# Autodesk Inventor assembly: RAI_Assembly
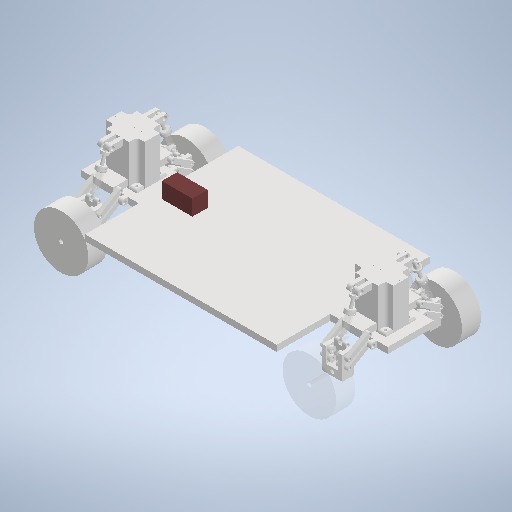
[picture p0: Inventor's stored thumbnail of the model, 512x512]
Saved by Autodesk Inventor 2025.2 (Build 292293000, 293)
## iProperties
Created: 2025-01-03
Part Number: RAI_Assembly
Document SubType Name: Assembly
Designer: SEON
Author: SEON
## Documents named in this file (15)
- C:\Users\SEON\Documents\Inventor\ProjectRAI\RAI_Assembly.iam
- C:\Users\SEON\Documents\Inventor\ProjectRAI\BottomFrame.ipt
- C:\Users\SEON\Documents\Inventor\ProjectRAI\SuspensionSupporter.ipt
- C:\Users\SEON\Documents\Inventor\ProjectRAI\TireDummy.ipt
- C:\Users\SEON\Documents\Inventor\ProjectRAI\SteeringFrame.ipt
- C:\Users\SEON\Documents\Inventor\ProjectRAI\SteeringConnector.ipt
- C:\Users\SEON\Documents\Inventor\ProjectRAI\SuspensionFrame.ipt
- C:\Users\SEON\Documents\Inventor\ProjectRAI\SuspensionAssembly.iam
- C:\Users\SEON\Documents\Inventor\ProjectRAI\SteeringFrameFront.ipt
- C:\Users\SEON\Documents\Inventor\ProjectRAI\Steering.ipt
- C:\Users\SEON\Documents\Inventor\ProjectRAI\996R_Servo.ipt
- C:\Users\SEON\Documents\Inventor\ProjectRAI\SteeringBase.ipt
- C:\Users\SEON\Documents\Inventor\ProjectRAI\SteeringAxis.ipt
- C:\Users\SEON\Documents\Inventor\ProjectRAI\DummyBallJoint.ipt
- C:\Users\SEON\Documents\Inventor\ProjectRAI\DummyBallJointF.ipt
## Components (64 placed, 14 different names)
1. BottomFrame:1 — 메이트:1, 메이트:2, 메이트:3, 메이트:5, 메이트:6, 메이트:17, 메이트:18, 메이트:21, 메이트:37, 메이트:43, 메이트:55, 메이트:62, 메이트:63, 메이트:64, 메이트:65, 메이트:67, 메이트:89, 메이트:91, 메이트:93, 메이트:111, 메이트:113, 메이트:115, 메이트:130, 메이트:152, 메이트:153, 메이트:154
2. SuspensionSupporter:1 — 메이트:1, 메이트:2, 메이트:3, 메이트:4, 메이트:46, 메이트:56, 메이트:146, 메이트:147, 메이트:149, 메이트:151
3. SuspensionSupporter:2 — 메이트:4, 메이트:5, 메이트:6, 메이트:23, 메이트:26, 메이트:35
4. TireDummy:1 — 메이트:7, 메이트:8
5. SteeringFrame:1 — 메이트:7, 메이트:8, 메이트:9, 메이트:10, 메이트:11, 메이트:12, 메이트:19, 메이트:24, 메이트:27, 메이트:28, 메이트:29, 메이트:30, 메이트:33, 메이트:34
6. SuspensionFrame:2 — 메이트:13, 메이트:14, 메이트:18, 메이트:21
7. SteeringConnector:3 — 메이트:9, 메이트:10, 메이트:13, 메이트:14
8. SteeringConnector:4 — 메이트:11, 메이트:12, 메이트:15, 메이트:16
9. SuspensionFrame:3 — 메이트:15, 메이트:16, 메이트:17
10. SuspensionFrame:4 — 메이트:19, 메이트:23, 메이트:31
11. SuspensionFrame:5 — 메이트:24, 메이트:26, 메이트:32
12. SteeringConnector:5 — 메이트:27, 메이트:28, 메이트:32
13. SteeringConnector:6 — 메이트:29, 메이트:30, 메이트:31
14. SuspensionAssembly:1 [sub-assembly] — 메이트:33, 메이트:34, 메이트:35
15. SuspensionFrame:6 — 메이트:44, 메이트:45, 메이트:46
16. SuspensionFrame:7 — 메이트:53, 메이트:54, 메이트:55
17. SuspensionFrame:8 — 메이트:36, 메이트:37, 메이트:42, 메이트:43
18. SuspensionFrame:9 — 메이트:51, 메이트:52, 메이트:56
19. SteeringFrame:2 — 메이트:36, 메이트:38, 메이트:39, 메이트:40, 메이트:41, 메이트:45, 메이트:47, 메이트:48, 메이트:49, 메이트:50, 메이트:60, 메이트:61, 메이트:148, 메이트:150
20. SteeringConnector:7 — 메이트:48, 메이트:49, 메이트:51, 메이트:52
21. SteeringConnector:8 — 메이트:38, 메이트:39, 메이트:44
22. SteeringConnector:9 — 메이트:47, 메이트:50, 메이트:53, 메이트:54
23. SteeringConnector:10 — 메이트:40, 메이트:41, 메이트:42
24. TireDummy:2 — 메이트:60, 메이트:61
25. SuspensionSupporter:3 — 메이트:62, 메이트:66, 메이트:67, 메이트:68, 메이트:69, 메이트:90, 메이트:92, 메이트:131
26. SuspensionSupporter:4 — 메이트:63, 메이트:64, 메이트:65, 메이트:66, 메이트:70, 메이트:71, 메이트:112, 메이트:114, 메이트:135, 메이트:136
27. SuspensionAssembly:3 [sub-assembly] — 메이트:68, 메이트:69, 메이트:129
28. SuspensionAssembly:4 [sub-assembly] — 메이트:70, 메이트:71, 메이트:125
29. SuspensionFrame:10 — 메이트:84, 메이트:85, 메이트:93, 메이트:127, 메이트:130
30. SuspensionFrame:11 — 메이트:82, 메이트:83, 메이트:90, 메이트:133
31. SuspensionFrame:12 — 메이트:86, 메이트:87, 메이트:92, 메이트:128, 메이트:131
32. SuspensionFrame:13 — 메이트:80, 메이트:81, 메이트:89, 메이트:91
33. SteeringConnector:11 — 메이트:86, 메이트:87
34. SteeringConnector:12 — 메이트:84, 메이트:85, 메이트:126
35. SteeringConnector:13 — 메이트:82, 메이트:83, 메이트:132
36. SteeringConnector:14 — 메이트:80, 메이트:81, 메이트:134
37. SuspensionFrame:14 — 메이트:113, 메이트:137
38. SuspensionFrame:15 — 메이트:112, 메이트:121, 메이트:135
39. SuspensionFrame:16 — 메이트:114, 메이트:136
40. SuspensionFrame:17 — 메이트:111, 메이트:115, 메이트:122
41. SteeringConnector:15 — 메이트:124
42. SteeringConnector:16 — 메이트:123
43. SteeringConnector:17 — 메이트:120
44. SteeringConnector:18
45. TireDummy:3 — 메이트:143, 메이트:144
46. TireDummy:4 — 메이트:140, 메이트:141
47. SteeringFrameFront:1 — 메이트:120, 메이트:121, 메이트:122, 메이트:123, 메이트:124, 메이트:125, 메이트:137, 메이트:142, 메이트:145
48. SteeringFrameFront:2 — 메이트:126, 메이트:127, 메이트:128, 메이트:129, 메이트:132, 메이트:133, 메이트:134, 메이트:138, 메이트:139
49. Steering:1 — 메이트:138, 메이트:139, 메이트:140, 메이트:141, 메이트:167, 메이트:168
50. Steering:2 — 메이트:142, 메이트:143, 메이트:144, 메이트:145, 메이트:165, 메이트:166
51. SuspensionAssembly:5 [sub-assembly] — 메이트:146, 메이트:147, 메이트:148
52. SuspensionAssembly:6 [sub-assembly] — 메이트:149, 메이트:150, 메이트:151
53. 996R_Servo:1 — 메이트:152, 메이트:153, 메이트:154, 메이트:155, 메이트:156
54. SteeringBase:1 — 메이트:155, 메이트:156, 메이트:161, 메이트:162, 메이트:163, 메이트:164
55. DummyBallJoint:1 — 메이트:161, 메이트:162, 접선:2
56. DummyBallJoint:2 — 메이트:163, 메이트:164, 접선:3
57. DummyBallJointF:1 — 메이트:169, 메이트:172, 접선:2
58. DummyBallJointF:2 — 메이트:170, 메이트:171, 접선:1
59. DummyBallJoint:3 — 메이트:165, 메이트:166, 접선:1
60. DummyBallJoint:4 — 메이트:167, 메이트:168, 접선:4
61. SteeringAxis:4 — 메이트:169, 메이트:170, 메이트:171, 메이트:172
62. DummyBallJointF:3 — 접선:4
63. DummyBallJointF:4 — 접선:3
64. SteeringAxis:5
## Relationships (148: Mate 144, Tangent 4)
- 메이트:1 [Mate]: BottomFrame:1 ↔ SuspensionSupporter:1
- 메이트:2 [Mate]: BottomFrame:1 ↔ SuspensionSupporter:1
- 메이트:3 [Mate]: BottomFrame:1 ↔ SuspensionSupporter:1
- 메이트:4 [Mate]: SuspensionSupporter:1 ↔ SuspensionSupporter:2
- 메이트:5 [Mate]: BottomFrame:1 ↔ SuspensionSupporter:2
- 메이트:6 [Mate]: BottomFrame:1 ↔ SuspensionSupporter:2
- 메이트:7 [Mate]: TireDummy:1 ↔ SteeringFrame:1
- 메이트:8 [Mate] (5 mm): TireDummy:1 ↔ SteeringFrame:1
- 메이트:9 [Mate]: SteeringFrame:1 ↔ SteeringConnector:3
- 메이트:10 [Mate]: SteeringFrame:1 ↔ SteeringConnector:3
- 메이트:11 [Mate]: SteeringFrame:1 ↔ SteeringConnector:4
- 메이트:12 [Mate]: SteeringFrame:1 ↔ SteeringConnector:4
- 메이트:13 [Mate]: SuspensionFrame:2 ↔ SteeringConnector:3
- 메이트:14 [Mate]: SuspensionFrame:2 ↔ SteeringConnector:3
- 메이트:15 [Mate]: SteeringConnector:4 ↔ SuspensionFrame:3
- 메이트:16 [Mate]: SteeringConnector:4 ↔ SuspensionFrame:3
- 메이트:17 [Mate]: BottomFrame:1 ↔ SuspensionFrame:3
- 메이트:18 [Mate]: BottomFrame:1 ↔ SuspensionFrame:2
- 메이트:19 [Mate]: SteeringFrame:1 ↔ SuspensionFrame:4
- 메이트:21 [Mate]: BottomFrame:1 ↔ SuspensionFrame:2
- 메이트:23 [Mate]: SuspensionSupporter:2 ↔ SuspensionFrame:4
- 메이트:24 [Mate]: SteeringFrame:1 ↔ SuspensionFrame:5
- 메이트:26 [Mate]: SuspensionSupporter:2 ↔ SuspensionFrame:5
- 메이트:27 [Mate]: SteeringFrame:1 ↔ SteeringConnector:5
- 메이트:28 [Mate]: SteeringFrame:1 ↔ SteeringConnector:5
- 메이트:29 [Mate]: SteeringFrame:1 ↔ SteeringConnector:6
- 메이트:30 [Mate]: SteeringFrame:1 ↔ SteeringConnector:6
- 메이트:31 [Mate]: SuspensionFrame:4 ↔ SteeringConnector:6
- 메이트:32 [Mate]: SuspensionFrame:5 ↔ SteeringConnector:5
- 메이트:33 [Mate]: SteeringFrame:1 ↔ SuspensionAssembly:1
- 메이트:34 [Mate]: SteeringFrame:1 ↔ SuspensionAssembly:1
- 메이트:35 [Mate]: SuspensionSupporter:2 ↔ SuspensionAssembly:1
- 메이트:36 [Mate]: SuspensionFrame:8 ↔ SteeringFrame:2
- 메이트:37 [Mate]: BottomFrame:1 ↔ SuspensionFrame:8
- 메이트:38 [Mate]: SteeringFrame:2 ↔ SteeringConnector:8
- 메이트:39 [Mate]: SteeringFrame:2 ↔ SteeringConnector:8
- 메이트:40 [Mate]: SteeringFrame:2 ↔ SteeringConnector:10
- 메이트:41 [Mate]: SteeringFrame:2 ↔ SteeringConnector:10
- 메이트:42 [Mate]: SuspensionFrame:8 ↔ SteeringConnector:10
- 메이트:43 [Mate]: BottomFrame:1 ↔ SuspensionFrame:8
- 메이트:44 [Mate]: SuspensionFrame:6 ↔ SteeringConnector:8
- 메이트:45 [Mate]: SuspensionFrame:6 ↔ SteeringFrame:2
- 메이트:46 [Mate]: SuspensionSupporter:1 ↔ SuspensionFrame:6
- 메이트:47 [Mate]: SteeringFrame:2 ↔ SteeringConnector:9
- 메이트:48 [Mate]: SteeringFrame:2 ↔ SteeringConnector:7
- 메이트:49 [Mate]: SteeringFrame:2 ↔ SteeringConnector:7
- 메이트:50 [Mate]: SteeringFrame:2 ↔ SteeringConnector:9
- 메이트:51 [Mate]: SuspensionFrame:9 ↔ SteeringConnector:7
- 메이트:52 [Mate]: SuspensionFrame:9 ↔ SteeringConnector:7
- 메이트:53 [Mate]: SuspensionFrame:7 ↔ SteeringConnector:9
- 메이트:54 [Mate]: SuspensionFrame:7 ↔ SteeringConnector:9
- 메이트:55 [Mate]: BottomFrame:1 ↔ SuspensionFrame:7
- 메이트:56 [Mate]: SuspensionSupporter:1 ↔ SuspensionFrame:9
- 메이트:60 [Mate]: SteeringFrame:2 ↔ TireDummy:2
- 메이트:61 [Mate] (5 mm): SteeringFrame:2 ↔ TireDummy:2
- 메이트:62 [Mate]: BottomFrame:1 ↔ SuspensionSupporter:3
- 메이트:63 [Mate]: BottomFrame:1 ↔ SuspensionSupporter:4
- 메이트:64 [Mate]: BottomFrame:1 ↔ SuspensionSupporter:4
- 메이트:65 [Mate]: BottomFrame:1 ↔ SuspensionSupporter:4
- 메이트:66 [Mate]: SuspensionSupporter:3 ↔ SuspensionSupporter:4
- 메이트:67 [Mate]: BottomFrame:1 ↔ SuspensionSupporter:3
- 메이트:68 [Mate]: SuspensionSupporter:3 ↔ SuspensionAssembly:3
- 메이트:69 [Mate]: SuspensionSupporter:3 ↔ SuspensionAssembly:3
- 메이트:70 [Mate]: SuspensionSupporter:4 ↔ SuspensionAssembly:4
- 메이트:71 [Mate]: SuspensionSupporter:4 ↔ SuspensionAssembly:4
- 메이트:80 [Mate]: SuspensionFrame:13 ↔ SteeringConnector:14
- 메이트:81 [Mate]: SuspensionFrame:13 ↔ SteeringConnector:14
- 메이트:82 [Mate]: SuspensionFrame:11 ↔ SteeringConnector:13
- 메이트:83 [Mate]: SuspensionFrame:11 ↔ SteeringConnector:13
- 메이트:84 [Mate]: SuspensionFrame:10 ↔ SteeringConnector:12
- 메이트:85 [Mate]: SuspensionFrame:10 ↔ SteeringConnector:12
- 메이트:86 [Mate]: SuspensionFrame:12 ↔ SteeringConnector:11
- 메이트:87 [Mate]: SuspensionFrame:12 ↔ SteeringConnector:11
- 메이트:89 [Mate]: BottomFrame:1 ↔ SuspensionFrame:13
- 메이트:90 [Mate]: SuspensionSupporter:3 ↔ SuspensionFrame:11
- 메이트:91 [Mate]: BottomFrame:1 ↔ SuspensionFrame:13
- 메이트:92 [Mate]: SuspensionSupporter:3 ↔ SuspensionFrame:12
- 메이트:93 [Mate]: BottomFrame:1 ↔ SuspensionFrame:10
- [Mate]: SuspensionFrame:17 ↔ SteeringConnector:18
- [Mate]: SuspensionFrame:17 ↔ SteeringConnector:18
- [Mate]: SuspensionFrame:15 ↔ SteeringConnector:17
- [Mate]: SuspensionFrame:15 ↔ SteeringConnector:17
- [Mate]: SuspensionFrame:14 ↔ SteeringConnector:16
- [Mate]: SuspensionFrame:14 ↔ SteeringConnector:16
- [Mate]: SuspensionFrame:16 ↔ SteeringConnector:15
- [Mate]: SuspensionFrame:16 ↔ SteeringConnector:15
- 메이트:111 [Mate]: BottomFrame:1 ↔ SuspensionFrame:17
- 메이트:112 [Mate]: SuspensionSupporter:4 ↔ SuspensionFrame:15
- 메이트:113 [Mate]: BottomFrame:1 ↔ SuspensionFrame:14
- 메이트:114 [Mate]: SuspensionSupporter:4 ↔ SuspensionFrame:16
- 메이트:115 [Mate]: BottomFrame:1 ↔ SuspensionFrame:17
- 메이트:120 [Mate]: SteeringConnector:17 ↔ SteeringFrameFront:1
- 메이트:121 [Mate]: SuspensionFrame:15 ↔ SteeringFrameFront:1
- 메이트:122 [Mate]: SuspensionFrame:17 ↔ SteeringFrameFront:1
- 메이트:123 [Mate]: SteeringConnector:16 ↔ SteeringFrameFront:1
- 메이트:124 [Mate]: SteeringConnector:15 ↔ SteeringFrameFront:1
- 메이트:125 [Mate]: SuspensionAssembly:4 ↔ SteeringFrameFront:1
- 메이트:126 [Mate]: SteeringConnector:12 ↔ SteeringFrameFront:2
- 메이트:127 [Mate]: SuspensionFrame:10 ↔ SteeringFrameFront:2
- 메이트:128 [Mate]: SuspensionFrame:12 ↔ SteeringFrameFront:2
- 메이트:129 [Mate]: SuspensionAssembly:3 ↔ SteeringFrameFront:2
- 메이트:130 [Mate]: BottomFrame:1 ↔ SuspensionFrame:10
- 메이트:131 [Mate]: SuspensionSupporter:3 ↔ SuspensionFrame:12
- 메이트:132 [Mate]: SteeringConnector:13 ↔ SteeringFrameFront:2
- 메이트:133 [Mate]: SuspensionFrame:11 ↔ SteeringFrameFront:2
- 메이트:134 [Mate]: SteeringConnector:14 ↔ SteeringFrameFront:2
- 메이트:135 [Mate]: SuspensionSupporter:4 ↔ SuspensionFrame:15
- 메이트:136 [Mate]: SuspensionSupporter:4 ↔ SuspensionFrame:16
- 메이트:137 [Mate]: SuspensionFrame:14 ↔ SteeringFrameFront:1
- 메이트:138 [Mate]: SteeringFrameFront:2 ↔ Steering:1
- 메이트:139 [Mate]: SteeringFrameFront:2 ↔ Steering:1
- 메이트:140 [Mate]: TireDummy:4 ↔ Steering:1
- 메이트:141 [Mate] (5 mm): TireDummy:4 ↔ Steering:1
- 메이트:142 [Mate]: SteeringFrameFront:1 ↔ Steering:2
- 메이트:143 [Mate]: TireDummy:3 ↔ Steering:2
- 메이트:144 [Mate] (5 mm): TireDummy:3 ↔ Steering:2
- 메이트:145 [Mate]: SteeringFrameFront:1 ↔ Steering:2
- 메이트:146 [Mate]: SuspensionSupporter:1 ↔ SuspensionAssembly:5
- 메이트:147 [Mate]: SuspensionSupporter:1 ↔ SuspensionAssembly:5
- 메이트:148 [Mate]: SteeringFrame:2 ↔ SuspensionAssembly:5
- 메이트:149 [Mate]: SuspensionSupporter:1 ↔ SuspensionAssembly:6
- 메이트:150 [Mate]: SteeringFrame:2 ↔ SuspensionAssembly:6
- 메이트:151 [Mate]: SuspensionSupporter:1 ↔ SuspensionAssembly:6
- 메이트:152 [Mate]: BottomFrame:1 ↔ 996R_Servo:1
- 메이트:153 [Mate]: BottomFrame:1 ↔ 996R_Servo:1
- 메이트:154 [Mate]: BottomFrame:1 ↔ 996R_Servo:1
- 메이트:155 [Mate]: 996R_Servo:1 ↔ SteeringBase:1
- 메이트:156 [Mate] (5 mm): 996R_Servo:1 ↔ SteeringBase:1
- 메이트:161 [Mate]: SteeringBase:1 ↔ DummyBallJoint:1
- 메이트:162 [Mate]: SteeringBase:1 ↔ DummyBallJoint:1
- 메이트:163 [Mate]: SteeringBase:1 ↔ DummyBallJoint:2
- 메이트:164 [Mate]: SteeringBase:1 ↔ DummyBallJoint:2
- 메이트:165 [Mate]: Steering:2 ↔ DummyBallJoint:3
- 메이트:166 [Mate]: Steering:2 ↔ DummyBallJoint:3
- 메이트:167 [Mate]: Steering:1 ↔ DummyBallJoint:4
- 메이트:168 [Mate]: Steering:1 ↔ DummyBallJoint:4
- 메이트:169 [Mate]: DummyBallJointF:1 ↔ SteeringAxis:4
- 메이트:170 [Mate]: DummyBallJointF:2 ↔ SteeringAxis:4
- 메이트:171 [Mate]: DummyBallJointF:2 ↔ SteeringAxis:4
- 메이트:172 [Mate]: DummyBallJointF:1 ↔ SteeringAxis:4
- [Mate]: DummyBallJointF:3 ↔ SteeringAxis:5
- [Mate]: DummyBallJointF:4 ↔ SteeringAxis:5
- [Mate]: DummyBallJointF:4 ↔ SteeringAxis:5
- [Mate]: DummyBallJointF:3 ↔ SteeringAxis:5
- 접선:1 [Tangent]: DummyBallJointF:2 ↔ DummyBallJoint:3
- 접선:2 [Tangent]: DummyBallJoint:1 ↔ DummyBallJointF:1
- 접선:3 [Tangent]: DummyBallJoint:2 ↔ DummyBallJointF:4
- 접선:4 [Tangent]: DummyBallJoint:4 ↔ DummyBallJointF:3
## Named parameters: d100_d84 = 0 mm, d101_d85 = 0 mm, d102_d86 = 0 mm, d103_d87 = 0 mm, d104_d88 = 0 mm, d105_d89 = 0 mm, d106_d90 = 0 mm, d107_d91 = 0 mm, d186_d182 = 0 mm, d187_d183 = 0 mm, d188_d184 = 0 mm, d189_d185 = 0 mm
